# Autodesk Inventor assembly: small rail assmb
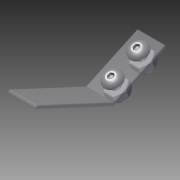
[picture p0: Inventor's stored thumbnail of the model, 180x180]
Saved by Autodesk Inventor 2014 SP1 (Build 180222100, 222)
## iProperties
Created: 2013-11-15
Part Number: small rail assmb
Document SubType Name: Assembly
Designer: RyanHughes
Author: RyanHughes
## Documents named in this file (4)
- C:\Users\Ryan\Desktop\sw\toss up 2ed A bot\intake\small rail assmb.iam
- C:\Users\Ryan\Desktop\sw\toss up 2ed A bot\intake\buckies poly\small rail.ipt
- C:\Users\Ryan\Desktop\sw\lib\Aperture VEX CAD Library\Hardware\8-32\8-32_.375.ipt
- C:\Users\Ryan\Desktop\sw\lib\Aperture VEX CAD Library\Hardware\8-32\8-32 Nylock.ipt
## Components (5 placed, 3 different names)
1. small rail:1 — Mate:1, Mate:2, Mate:3, Mate:4, Mate:5
2. 8-32_.375:1 — Mate:1, Mate:2, Mate:6
3. 8-32_.375:2 — Mate:3, Mate:4, Mate:7
4. 8-32 Nylock:1 — Mate:5, Mate:6, Flush:1
5. 8-32 Nylock:2 — Mate:7, Flush:1
## Relationships (8: Mate 7, Flush 1)
- Mate:1: small rail:1 ↔ 8-32_.375:1
- Mate:2: small rail:1 ↔ 8-32_.375:1
- Mate:3: small rail:1 ↔ 8-32_.375:2
- Mate:4: small rail:1 ↔ 8-32_.375:2
- Mate:5 (1.5875 mm): small rail:1 ↔ 8-32 Nylock:1
- Mate:6: 8-32_.375:1 ↔ 8-32 Nylock:1
- Mate:7: 8-32_.375:2 ↔ 8-32 Nylock:2
- Flush:1: 8-32 Nylock:1 ↔ 8-32 Nylock:2
